# Autodesk Inventor assembly: Base 03
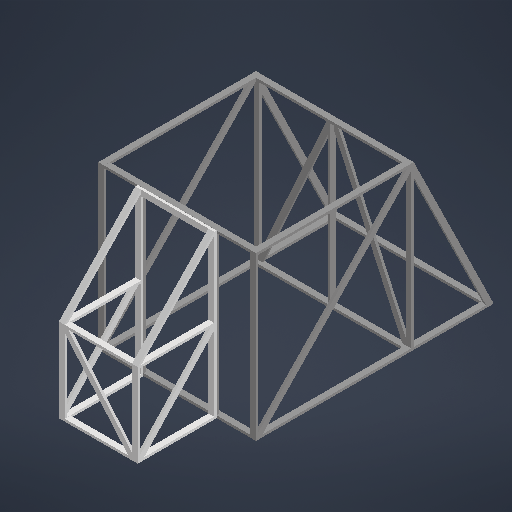
[picture p0: Inventor's stored thumbnail of the model, 512x512]
Saved by Autodesk Inventor 2026 (Build 300175000, 175)
## iProperties
Created: 2024-09-19
Part Number: Base 03
Document SubType Name: Assembly
Designer: User
Author: User
## Documents named in this file (13)
- C:\Users\trott\Documents\UofSC-ASME-Tiger-Burn-Design-2025\CAD\Body\Base 03\Base 03.iam
- C:\Users\trott\Documents\UofSC-ASME-Tiger-Burn-Design-2025\CAD\Body\Base 03\2x4x144.ipt
- C:\Users\trott\Documents\UofSC-ASME-Tiger-Burn-Design-2025\CAD\Body\Base 03\2x4x89.ipt
- C:\Users\trott\Documents\UofSC-ASME-Tiger-Burn-Design-2025\CAD\Body\Base 03\2x4x96.ipt
- C:\Users\trott\Documents\UofSC-ASME-Tiger-Burn-Design-2025\CAD\Body\Base 03\S_2x4x105.499.ipt
- C:\Users\trott\Documents\UofSC-ASME-Tiger-Burn-Design-2025\CAD\Body\Base 03\S_2x4x133.660.ipt
- C:\Users\trott\Documents\UofSC-ASME-Tiger-Burn-Design-2025\CAD\Body\Base 03\S_2x4x108.675.ipt
- C:\Users\trott\Documents\UofSC-ASME-Tiger-Burn-Design-2025\CAD\Body\Base 03\2x4x41.ipt
- C:\Users\trott\Documents\UofSC-ASME-Tiger-Burn-Design-2025\CAD\Body\Base 03\2x4x44.5.ipt
- C:\Users\trott\Documents\UofSC-ASME-Tiger-Burn-Design-2025\CAD\Body\Base 03\S_2x4x66.83.ipt
- C:\Users\trott\Documents\UofSC-ASME-Tiger-Burn-Design-2025\CAD\Body\Base 03\S_2x4x65.795.ipt
- C:\Users\trott\Documents\UofSC-ASME-Tiger-Burn-Design-2025\CAD\Body\Base 03\S_2x4x63.127.ipt
- C:\Users\trott\Documents\UofSC-ASME-Tiger-Burn-Design-2025\CAD\Body\Base 03\2x4x48.ipt
## Components (40 placed, 12 different names)
1. 2x4x144:1 — Flush:3, Flush:4, Flush:5, Mate:2, Mate:3, Mate:5, Flush:15, Flush:16, Flush:17, Flush:38
2. 2x4x144:2 — Flush:3, Flush:4, Flush:5, Mate:1, Flush:6, Flush:7, Flush:8, Flush:9, Flush:10, Mate:4, Mate:6, Flush:12, Flush:13, Flush:14, Mate:24
3. 2x4x89:1 — Mate:1, Flush:6, Flush:7, Flush:11, Mate:46, Mate:50
4. 2x4x89:2 — Flush:10, Flush:11, Flush:18, Flush:19, Mate:11, Flush:28
5. 2x4x89:3 — Flush:8, Flush:9, Mate:2
6. 2x4x96:1 — Mate:4, Flush:13, Flush:14, Mate:8, Flush:21, Flush:22, Flush:36
7. 2x4x96:2 — Mate:3, Flush:15, Flush:16, Mate:7, Flush:20, Flush:23
8. 2x4x96:3 — Mate:5, Flush:17, Flush:18, Flush:31, Mate:22
9. 2x4x96:4 — Mate:6, Flush:12, Flush:19, Mate:23, Flush:39
10. 2x4x96:5 — Mate:8, Flush:21, Flush:22, Mate:9, Flush:26, Mate:10, Flush:27
11. 2x4x96:6 — Mate:7, Flush:20, Flush:23, Flush:24, Flush:25, Mate:21, Flush:37
12. 2x4x89:4 — Flush:24, Mate:10, Flush:27, Mate:35, Flush:63, Mate:44, Flush:80, Flush:82
13. 2x4x89:5 — Flush:25, Mate:9, Flush:26, Mate:18, Mate:20
14. 2x4x96:8 — Mate:11, Flush:28, Flush:31, Mate:17, Flush:34, Mate:19, Flush:35
15. S_2x4x105.499:3 — Mate:17, Mate:18, Flush:34
16. S_2x4x105.499:4 — Mate:19, Mate:20, Flush:35
17. S_2x4x133.660:1 — Flush:36
18. S_2x4x133.660:2 — Mate:21, Mate:22, Flush:37
19. S_2x4x108.675:1 — Flush:38
20. S_2x4x108.675:2 — Mate:23, Mate:24, Flush:39
21. 2x4x41:1 — Mate:47
22. 2x4x41:2 — Mate:58
23. 2x4x44.5:1 — Flush:61, Flush:62
24. S_2x4x66.83:1 — Flush:61, Mate:56
25. 2x4x96:1 — Mate:35, Flush:62, Flush:63, Mate:52, Mate:55, Flush:78
26. S_2x4x65.795:1
27. S_2x4x65.795:2
28. S_2x4x63.127:1
29. 2x4x44.5:2 — Flush:74
30. 2x4x96:10 — Mate:44, Mate:49, Mate:57, Flush:79, Flush:81, Mate:59
31. S_2x4x66.83:2 — Flush:74
32. 2x4x48:1 — Mate:46, Flush:76, Flush:77, Mate:48
33. 2x4x48:2 — Mate:47, Flush:76, Flush:77
34. 2x4x48:3 — Mate:48, Mate:49
35. 2x4x48:4 — Mate:50, Mate:51, Mate:53, Mate:54
36. 2x4x48:5 — Mate:51, Mate:52
37. 2x4x48:6 — Mate:53, Mate:54
38. 2x4x48:7 — Mate:55, Mate:56, Flush:78
39. 2x4x48:8 — Mate:57, Mate:58, Flush:79
40. 2x4x48:9 — Flush:80, Flush:81, Mate:59, Flush:82
## Relationships (79: Flush 44, Mate 35)
- Flush:3 (2349.5 mm): 2x4x144:1 ↔ 2x4x144:2
- Flush:4: 2x4x144:1 ↔ 2x4x144:2
- Flush:5: 2x4x144:1 ↔ 2x4x144:2
- Mate:1: 2x4x144:2 ↔ 2x4x89:1
- Flush:6: 2x4x144:2 ↔ 2x4x89:1
- Flush:7: 2x4x144:2 ↔ 2x4x89:1
- Flush:8: 2x4x144:2 ↔ 2x4x89:3
- Flush:9: 2x4x144:2 ↔ 2x4x89:3
- Mate:2: 2x4x144:1 ↔ 2x4x89:3
- Flush:10: 2x4x144:2 ↔ 2x4x89:2
- Flush:11 (2349.5 mm): 2x4x89:1 ↔ 2x4x89:2
- Mate:3: 2x4x144:1 ↔ 2x4x96:2
- Mate:4: 2x4x144:2 ↔ 2x4x96:1
- Mate:5: 2x4x144:1 ↔ 2x4x96:3
- Mate:6: 2x4x144:2 ↔ 2x4x96:4
- Flush:12: 2x4x144:2 ↔ 2x4x96:4
- Flush:13: 2x4x144:2 ↔ 2x4x96:1
- Flush:14: 2x4x144:2 ↔ 2x4x96:1
- Flush:15: 2x4x144:1 ↔ 2x4x96:2
- Flush:16: 2x4x144:1 ↔ 2x4x96:2
- Flush:17: 2x4x144:1 ↔ 2x4x96:3
- Flush:18: 2x4x89:2 ↔ 2x4x96:3
- Flush:19: 2x4x89:2 ↔ 2x4x96:4
- Mate:7: 2x4x96:2 ↔ 2x4x96:6
- Mate:8: 2x4x96:1 ↔ 2x4x96:5
- Flush:20: 2x4x96:2 ↔ 2x4x96:6
- Flush:21: 2x4x96:1 ↔ 2x4x96:5
- Flush:22: 2x4x96:1 ↔ 2x4x96:5
- Flush:23: 2x4x96:2 ↔ 2x4x96:6
- Flush:24: 2x4x96:6 ↔ 2x4x89:4
- Flush:25: 2x4x96:6 ↔ 2x4x89:5
- Mate:9: 2x4x96:5 ↔ 2x4x89:5
- Flush:26: 2x4x96:5 ↔ 2x4x89:5
- Mate:10: 2x4x96:5 ↔ 2x4x89:4
- Flush:27: 2x4x96:5 ↔ 2x4x89:4
- Mate:11: 2x4x89:2 ↔ 2x4x96:8
- Flush:28: 2x4x89:2 ↔ 2x4x96:8
- Flush:31 (1200.15 mm): 2x4x96:3 ↔ 2x4x96:8
- Mate:17: 2x4x96:8 ↔ S_2x4x105.499:3
- Mate:18: 2x4x89:5 ↔ S_2x4x105.499:3
- Flush:34: 2x4x96:8 ↔ S_2x4x105.499:3
- Mate:19: 2x4x96:8 ↔ S_2x4x105.499:4
- Mate:20: 2x4x89:5 ↔ S_2x4x105.499:4
- Flush:35: 2x4x96:8 ↔ S_2x4x105.499:4
- Flush:36: 2x4x96:1 ↔ S_2x4x133.660:1
- Mate:21: 2x4x96:6 ↔ S_2x4x133.660:2
- Mate:22: 2x4x96:3 ↔ S_2x4x133.660:2
- Flush:37: 2x4x96:6 ↔ S_2x4x133.660:2
- Flush:38: 2x4x144:1 ↔ S_2x4x108.675:1
- Mate:23: 2x4x96:4 ↔ S_2x4x108.675:2
- Mate:24: 2x4x144:2 ↔ S_2x4x108.675:2
- Flush:39: 2x4x96:4 ↔ S_2x4x108.675:2
- Flush:61: 2x4x44.5:1 ↔ S_2x4x66.83:1
- Mate:35: 2x4x89:4 ↔ 2x4x96:1
- Flush:62: 2x4x44.5:1 ↔ 2x4x96:1
- Flush:63: 2x4x89:4 ↔ 2x4x96:1
- Mate:44: 2x4x89:4 ↔ 2x4x96:10
- Flush:74: 2x4x44.5:2 ↔ S_2x4x66.83:2
- Mate:46: 2x4x89:1 ↔ 2x4x48:1
- Mate:47: 2x4x41:1 ↔ 2x4x48:2
- Flush:76: 2x4x48:1 ↔ 2x4x48:2
- Flush:77: 2x4x48:1 ↔ 2x4x48:2
- Mate:48: 2x4x48:1 ↔ 2x4x48:3
- Mate:49: 2x4x96:10 ↔ 2x4x48:3
- Mate:50: 2x4x89:1 ↔ 2x4x48:4
- Mate:51: 2x4x48:4 ↔ 2x4x48:5
- Mate:52: 2x4x96:1 ↔ 2x4x48:5
- Mate:53: 2x4x48:4 ↔ 2x4x48:6
- Mate:54: 2x4x48:4 ↔ 2x4x48:6
- Mate:55: 2x4x96:1 ↔ 2x4x48:7
- Mate:56: S_2x4x66.83:1 ↔ 2x4x48:7
- Flush:78: 2x4x96:1 ↔ 2x4x48:7
- Mate:57: 2x4x96:10 ↔ 2x4x48:8
- Mate:58: 2x4x41:2 ↔ 2x4x48:8
- Flush:79: 2x4x96:10 ↔ 2x4x48:8
- Flush:80: 2x4x89:4 ↔ 2x4x48:9
- Flush:81: 2x4x96:10 ↔ 2x4x48:9
- Mate:59: 2x4x96:10 ↔ 2x4x48:9
- Flush:82: 2x4x89:4 ↔ 2x4x48:9
